# Autodesk Inventor assembly: motor sub assembley
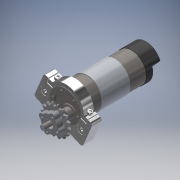
[picture p0: Inventor's stored thumbnail of the model, 180x180]
Saved by Autodesk Inventor 2017 (Build 210142000, 142)
## iProperties
Created: 2017-08-09
Part Number: motor sub assembley
Document SubType Name: Assembly
Designer: User
Author: User
## Documents named in this file (5)
- C:\Robotics\CAD\2016-17_CAD\DriveTrain\motor sub assembley.iam
- C:\Robotics\CAD\COTSParts\Actobotics\am-3102NeveRest20 (1).ipt
- C:\Robotics\CAD\COTSParts\Tetrix\tetrix-motor-mounts-1.snapshot.1\Tetrex 2pc motor mount.ipt
- C:\Robotics\CAD\COTSParts\Actobotics\615 parts\615102.ipt
- C:\Robotics\CAD\COTSParts\Actobotics\545 parts\545556.ipt
## Components (4 placed, 4 different names)
1. am-3102NeveRest20 (1):1 — Mate:1, Mate:2, Mate:3
2. Tetrex 2pc motor mount:1 — Mate:1
3. 615102:1 — Mate:2, Insert:1
4. 545556:1 — Mate:3, Insert:1
## Relationships (4: Mate 3, Insert 1)
- Mate:1: am-3102NeveRest20 (1):1 ↔ Tetrex 2pc motor mount:1
- Mate:2: am-3102NeveRest20 (1):1 ↔ 615102:1
- Mate:3: am-3102NeveRest20 (1):1 ↔ 545556:1
- Insert:1: 615102:1 ↔ 545556:1
